# Autodesk Inventor assembly: AS-070S-0250-10
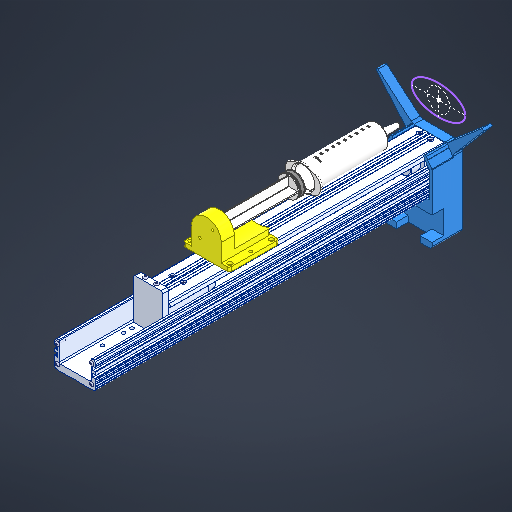
[picture p0: Inventor's stored thumbnail of the model, 512x512]
Saved by Autodesk Inventor 2027 (Build 310192060, 192F)
## iProperties
Created: 2018-09-27
Part Number: AS-070S-0250-10
Description: STEP AP214
Document SubType Name: Assembly
Designer: trtrn
Sending System: SolidWorks 2014
Preprocessor: SwSTEP 2.0
Title: AS-070S-0250-10.STEP
Author: user
Revision Number: ANY
## Documents named in this file (7)
- G:\My Drive\Project\GLUE01\Cad\PA1\AS-070S-0250-10\AS-070S-0250-10.iam
- G:\My Drive\Project\GLUE01\Cad\PA1\AS-070S-0250-10\AS-070S-0250 MAIN BASE.ipt
- G:\My Drive\Project\GLUE01\Cad\PA1\AS-070S-0250-10\TRUSS M4x10L-2_Ç¥ÁØ.ipt
- G:\My Drive\Project\GLUE01\Cad\PA1\AS-070S-0250-10\AS-070-SLIDER.ipt
- G:\My Drive\Project\GLUE01\Cad\PA1\Dam1.ipt
- G:\My Drive\Project\GLUE01\Cad\PA1\KeChan.ipt
- G:\My Drive\Project\GLUE01\Cad\PA1\Syringe_100ml.ipt
## Components (15 placed, 15 different names)
1. AS-070S-0250 MAIN BASE_1 — Mate:1, Angle:1, Mate:2, Mate:16, Tangent:1, Angle:3, Flush:1
2. TRUSS M4x10L-2_Ç¥ÁØ_4
3. TRUSS M4x10L-2_Ç¥ÁØ_6
4. TRUSS M4x10L-2_Ç¥ÁØ_7
5. TRUSS M4x10L-2_Ç¥ÁØ_11
6. TRUSS M4x10L-2_Ç¥ÁØ_13
7. TRUSS M4x10L-2_Ç¥ÁØ_14
8. TRUSS M4x10L-2_Ç¥ÁØ_18
9. TRUSS M4x10L-2_Ç¥ÁØ_19
10. TRUSS M4x10L-2_Ç¥ÁØ_20
11. AS-070-SLIDER_21 — Mate:1, Angle:1, Mate:2, Mate:3, Mate:4, Mate:5, Mate:6, Mate:7, Mate:15
12. Dam1:1 — Mate:3, Mate:4, Mate:5, Mate:6, Mate:7, Mate:13, Mate:14, Angle:2, Mate:15
13. KeChan:1 — Mate:16, Tangent:1, Angle:3, Flush:1
14. Syringe_100ml:1 — Mate:13, Mate:14, Angle:2
15. TRUSS M4x10L-2_Ç¥ÁØ_12
## Relationships (16: Mate 11, Angle 3, Tangent 1, Flush 1)
- Mate:1: AS-070S-0250 MAIN BASE_1 ↔ AS-070-SLIDER_21
- Angle:1 (0 deg): AS-070S-0250 MAIN BASE_1 ↔ AS-070-SLIDER_21
- Mate:2: AS-070S-0250 MAIN BASE_1 ↔ AS-070-SLIDER_21
- Mate:3: AS-070-SLIDER_21 ↔ Dam1:1
- Mate:4: AS-070-SLIDER_21 ↔ Dam1:1
- Mate:5: AS-070-SLIDER_21 ↔ Dam1:1
- Mate:6: AS-070-SLIDER_21 ↔ Dam1:1
- Mate:7: AS-070-SLIDER_21 ↔ Dam1:1
- Mate:13: Dam1:1 ↔ Syringe_100ml:1
- Mate:14: Dam1:1 ↔ Syringe_100ml:1
- Angle:2 (0 deg): Dam1:1 ↔ Syringe_100ml:1
- Mate:15: AS-070-SLIDER_21 ↔ Dam1:1
- Mate:16: AS-070S-0250 MAIN BASE_1 ↔ KeChan:1
- Tangent:1: AS-070S-0250 MAIN BASE_1 ↔ KeChan:1
- Angle:3 (0 deg): AS-070S-0250 MAIN BASE_1 ↔ KeChan:1
- Flush:1 (-5 mm): AS-070S-0250 MAIN BASE_1 ↔ KeChan:1
